# Autodesk Inventor assembly: mt4008_Act_Ver8
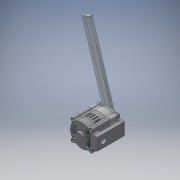
[picture p0: Inventor's stored thumbnail of the model, 180x180]
Saved by Autodesk Inventor 2019.3 (Build 233278000, 278)
## iProperties
Created: 2019-06-20
Part Number: mt4008_Act_Ver8
Document SubType Name: Assembly
Designer: cdi
Author: cdi
## Documents named in this file (20)
- C:\Users\cdi\SynologyDrive\workspace_inventor\2019_06_19.MT4008_actuator\[github_upload]\3d_print_planetary_gear\inventor_file\mt4008_Act_Ver8.iam
- C:\Users\cdi\SynologyDrive\workspace_inventor\2019_06_19.MT4008_actuator\[github_upload]\3d_print_planetary_gear\inventor_file\tarot-mt4008-motor-1.snapshot.3\inventor_export\Tarot 4008 Motor Assembly.iam
- C:\Users\cdi\SynologyDrive\workspace_inventor\2019_06_19.MT4008_actuator\[github_upload]\3d_print_planetary_gear\inventor_file\AS5147_3D_Export\Inventor_AS5147_ENC_ANGLE_VER01\AS5147_ENC_ANGLE_VER01.iam
- C:\Users\cdi\SynologyDrive\workspace_inventor\2019_06_19.MT4008_actuator\[github_upload]\3d_print_planetary_gear\inventor_file\motor_and_magnet_holder.ipt
- C:\Users\cdi\SynologyDrive\workspace_inventor\2019_06_19.MT4008_actuator\[github_upload]\3d_print_planetary_gear\inventor_file\magnet_6_2.5.ipt
- C:\Users\cdi\SynologyDrive\workspace_inventor\2019_06_19.MT4008_actuator\[github_upload]\3d_print_planetary_gear\inventor_file\bearing_52_40_7.ipt
- C:\Users\cdi\SynologyDrive\workspace_inventor\2019_06_19.MT4008_actuator\[github_upload]\3d_print_planetary_gear\inventor_file\pin_3_22.ipt
- C:\Users\cdi\SynologyDrive\workspace_inventor\2019_06_19.MT4008_actuator\[github_upload]\3d_print_planetary_gear\inventor_file\outer_bearing_holder_new.ipt
- C:\Users\cdi\SynologyDrive\workspace_inventor\2019_06_19.MT4008_actuator\[github_upload]\3d_print_planetary_gear\inventor_file\sun_gear_m0.65_T10.ipt
- C:\Users\cdi\SynologyDrive\workspace_inventor\2019_06_19.MT4008_actuator\[github_upload]\3d_print_planetary_gear\inventor_file\planet_gear_design\Design Accelerator\ver7\ring_gear_m0.65_T70.ipt
- C:\Users\cdi\SynologyDrive\workspace_inventor\2019_06_19.MT4008_actuator\[github_upload]\3d_print_planetary_gear\inventor_file\planet_gear_design\Design Accelerator\ver7\planet_gear_m0.65_T30.ipt
- C:\Users\cdi\SynologyDrive\workspace_inventor\2019_06_19.MT4008_actuator\[github_upload]\3d_print_planetary_gear\inventor_file\carrier_cover_14.344.ipt
- C:\Users\cdi\SynologyDrive\workspace_inventor\2019_06_19.MT4008_actuator\[github_upload]\3d_print_planetary_gear\inventor_file\carrier_gear_hold_14.344.ipt
- C:\Users\cdi\SynologyDrive\workspace_inventor\2019_06_19.MT4008_actuator\[github_upload]\3d_print_planetary_gear\inventor_file\sun_gear_adapter_withfan.ipt
- C:\Users\cdi\SynologyDrive\workspace_inventor\2019_06_19.MT4008_actuator\[github_upload]\3d_print_planetary_gear\inventor_file\motor_mount_with_motor_driver.ipt
- C:\Users\cdi\SynologyDrive\workspace_inventor\2019_06_19.MT4008_actuator\[github_upload]\3d_print_planetary_gear\inventor_file\motor_fixer_with_motor_driver.ipt
- C:\Users\cdi\SynologyDrive\workspace_inventor\2019_06_19.MT4008_actuator\[github_upload]\3d_print_planetary_gear\inventor_file\bearing_32_20_7_.ipt
- C:\Users\cdi\SynologyDrive\workspace_inventor\2019_06_19.MT4008_actuator\[github_upload]\3d_print_planetary_gear\inventor_file\test_arm_2.ipt
- C:\Users\cdi\SynologyDrive\workspace_inventor\2019_06_19.MT4008_actuator\[github_upload]\3d_print_planetary_gear\inventor_file\MJVESC_CIR_3D_Export\inv\MJVESC_MINI_VER03.ipt
- C:\Users\cdi\SynologyDrive\workspace_inventor\2019_06_19.MT4008_actuator\[github_upload]\3d_print_planetary_gear\inventor_file\as5047_holder_adder.ipt
## Components (20 placed, 19 different names)
1. Tarot 4008 Motor Assembly:1 [sub-assembly] — Mate:1, Mate:3, Mate:5, Mate:169, Mate:170, 메이트:173, 메이트:174
2. AS5147_ENC_ANGLE_VER01:1 [sub-assembly] — Mate:1, Mate:205, Mate:206, Mate:208
3. motor_and_magnet_holder:1 — Mate:2, Mate:3, Mate:4, Mate:5
4. magnet_6_2.5:1 — Mate:2, Mate:4
5. bearing_52_40_7:1 — Mate:148, Mate:160, 메이트:177, 메이트:178
6. pin_3_22:1 — Mate:158, Mate:159, Mate:161
7. sun_gear_m0.65_T10:1 — Mate:148, Mate:157, Mate:171, Mate:172
8. carrier_gear_hold_14.344:1 — Mate:155, Mate:156, Mate:157, Mate:158, Mate:159, Mate:160, Mate:162, Mate:163
9. planet_gear_m0.65_T30:1 — Mate:155, Mate:156
10. ring_gear_m0.65_T70:1 — Mate:154, Mate:166, Mate:167, 메이트:176, 메이트:179, 메이트:180
11. bearing_52_40_7:2 — Mate:143, Mate:154, Mate:164
12. carrier_cover_14.344:1 — Mate:161, Mate:162, Mate:163, Mate:164, 플러쉬:1, 메이트:199
13. outer_bearing_holder_new:1 — Mate:143, Mate:166, Mate:167, 각도:1
14. sun_gear_adapter_withfan:1 — Mate:169, Mate:170, Mate:171, Mate:172
15. motor_mount_with_motor_driver:1 — 메이트:173, 메이트:174, 메이트:175, 메이트:176, 메이트:177, 메이트:178, 메이트:179, 메이트:180, 메이트:190, 메이트:191, 메이트:192, Mate:202, Mate:203, Mate:204, Mate:207, Mate:209
16. motor_fixer_with_motor_driver:1 — 메이트:190, 메이트:191, 메이트:192, 메이트:195, 메이트:196
17. bearing_32_20_7_:1 — 메이트:195, 메이트:196
18. test_arm_2:1 — 플러쉬:1, 메이트:199
19. MJVESC_MINI_VER03:1 — Mate:202, Mate:203, Mate:204
20. as5047_holder_adder:1 — Mate:205, Mate:206, Mate:207, Mate:208, Mate:209
## Relationships (48: Mate 46, Angle 1, Flush 1)
- Mate:1: Tarot 4008 Motor Assembly:1 ↔ AS5147_ENC_ANGLE_VER01:1
- Mate:2: motor_and_magnet_holder:1 ↔ magnet_6_2.5:1
- Mate:3: Tarot 4008 Motor Assembly:1 ↔ motor_and_magnet_holder:1
- Mate:4: motor_and_magnet_holder:1 ↔ magnet_6_2.5:1
- Mate:5: Tarot 4008 Motor Assembly:1 ↔ motor_and_magnet_holder:1
- Mate:143: bearing_52_40_7:2 ↔ outer_bearing_holder_new:1
- Mate:148: bearing_52_40_7:1 ↔ sun_gear_m0.65_T10:1
- Mate:154: ring_gear_m0.65_T70:1 ↔ bearing_52_40_7:2
- Mate:155: carrier_gear_hold_14.344:1 ↔ planet_gear_m0.65_T30:1
- Mate:156: carrier_gear_hold_14.344:1 ↔ planet_gear_m0.65_T30:1
- Mate:157: sun_gear_m0.65_T10:1 ↔ carrier_gear_hold_14.344:1
- Mate:158: pin_3_22:1 ↔ carrier_gear_hold_14.344:1
- Mate:159: pin_3_22:1 ↔ carrier_gear_hold_14.344:1
- Mate:160: bearing_52_40_7:1 ↔ carrier_gear_hold_14.344:1
- Mate:161: pin_3_22:1 ↔ carrier_cover_14.344:1
- Mate:162: carrier_gear_hold_14.344:1 ↔ carrier_cover_14.344:1
- Mate:163: carrier_gear_hold_14.344:1 ↔ carrier_cover_14.344:1
- Mate:164: bearing_52_40_7:2 ↔ carrier_cover_14.344:1
- Mate:166: ring_gear_m0.65_T70:1 ↔ outer_bearing_holder_new:1
- Mate:167: ring_gear_m0.65_T70:1 ↔ outer_bearing_holder_new:1
- Mate:169: Tarot 4008 Motor Assembly:1 ↔ sun_gear_adapter_withfan:1
- Mate:170: Tarot 4008 Motor Assembly:1 ↔ sun_gear_adapter_withfan:1
- Mate:171: sun_gear_m0.65_T10:1 ↔ sun_gear_adapter_withfan:1
- Mate:172: sun_gear_m0.65_T10:1 ↔ sun_gear_adapter_withfan:1
- 메이트:173 [Mate]: Tarot 4008 Motor Assembly:1 ↔ motor_mount_with_motor_driver:1
- 메이트:174 [Mate]: Tarot 4008 Motor Assembly:1 ↔ motor_mount_with_motor_driver:1
- 메이트:175 [Mate]: motor_mount_with_motor_driver:1
- 메이트:176 [Mate]: ring_gear_m0.65_T70:1 ↔ motor_mount_with_motor_driver:1
- 메이트:177 [Mate]: bearing_52_40_7:1 ↔ motor_mount_with_motor_driver:1
- 메이트:178 [Mate]: bearing_52_40_7:1 ↔ motor_mount_with_motor_driver:1
- 메이트:179 [Mate]: ring_gear_m0.65_T70:1 ↔ motor_mount_with_motor_driver:1
- 메이트:180 [Mate]: ring_gear_m0.65_T70:1 ↔ motor_mount_with_motor_driver:1
- 각도:1 [Angle] (0 deg): outer_bearing_holder_new:1
- 메이트:190 [Mate]: motor_mount_with_motor_driver:1 ↔ motor_fixer_with_motor_driver:1
- 메이트:191 [Mate]: motor_mount_with_motor_driver:1 ↔ motor_fixer_with_motor_driver:1
- 메이트:192 [Mate]: motor_mount_with_motor_driver:1 ↔ motor_fixer_with_motor_driver:1
- 메이트:195 [Mate]: motor_fixer_with_motor_driver:1 ↔ bearing_32_20_7_:1
- 메이트:196 [Mate]: motor_fixer_with_motor_driver:1 ↔ bearing_32_20_7_:1
- 플러쉬:1 [Flush]: carrier_cover_14.344:1 ↔ test_arm_2:1
- 메이트:199 [Mate]: carrier_cover_14.344:1 ↔ test_arm_2:1
- Mate:202: motor_mount_with_motor_driver:1 ↔ MJVESC_MINI_VER03:1
- Mate:203: motor_mount_with_motor_driver:1 ↔ MJVESC_MINI_VER03:1
- Mate:204: motor_mount_with_motor_driver:1 ↔ MJVESC_MINI_VER03:1
- Mate:205: AS5147_ENC_ANGLE_VER01:1 ↔ as5047_holder_adder:1
- Mate:206: AS5147_ENC_ANGLE_VER01:1 ↔ as5047_holder_adder:1
- Mate:207: motor_mount_with_motor_driver:1 ↔ as5047_holder_adder:1
- Mate:208: AS5147_ENC_ANGLE_VER01:1 ↔ as5047_holder_adder:1
- Mate:209: motor_mount_with_motor_driver:1 ↔ as5047_holder_adder:1
